# Autodesk Inventor assembly: 軸受け下の図面用
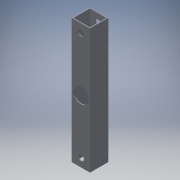
[picture p0: Inventor's stored thumbnail of the model, 180x180]
Saved by Autodesk Inventor 2018 (Build 220112000, 112)
## iProperties
Created: 2017-09-15
Part Number: 軸受け下の図面用
Material: 一般
Document SubType Name: Assembly
Designer: Kenta
Author: Kenta
## Documents named in this file (2)
- C:\Users\Kenta\Documents\workspace\rbbr\cart\シャーシ改でアッカーマン検討\軸受け下の図面用.iam
- C:\Users\Kenta\Documents\workspace\rbbr\cart\前足改\軸受下用.ipt
## Components (2 placed, 1 different names)
1. 軸受下用:1 — リジッド:1
2. 軸受下用:2 — リジッド:1
## Relationships (1: WeldJoint 1)
- リジッド:1 [WeldJoint]: 軸受下用:1 ↔ 軸受下用:2
